# Autodesk Inventor assembly: segment2
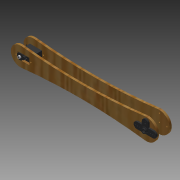
[picture p0: Inventor's stored thumbnail of the model, 180x180]
Saved by Autodesk Inventor 2013 (Build 170138000, 138)
## iProperties
Created: 2014-10-09
Part Number: segment2
Document SubType Name: Assembly
Designer: Masta
Author: Masta
## Documents named in this file (4)
- D:\DrOctopus\3D model\segment2.iam
- D:\DrOctopus\3D model\servo arm BMS-630MG tripple.ipt
- D:\DrOctopus\3D model\segment2a.ipt
- D:\DrOctopus\3D model\serwo 2.8kg DS939HV.ipt
## Components (4 placed, 3 different names)
1. servo arm BMS-630MG tripple:1 — Insert:1, Insert:2
2. segment2a:1 — Insert:1, Insert:2, Insert:3, Insert:4, Insert:5, Tangent:1
3. serwo 2.8kg DS939HV:1 — Insert:3, Insert:4
4. segment2a:2 — Insert:5, Tangent:1
## Relationships (6: Insert 5, Tangent 1)
- Insert:1: servo arm BMS-630MG tripple:1 ↔ segment2a:1
- Insert:2: servo arm BMS-630MG tripple:1 ↔ segment2a:1
- Insert:3 (2 mm): segment2a:1 ↔ serwo 2.8kg DS939HV:1
- Insert:4 (2 mm): segment2a:1 ↔ serwo 2.8kg DS939HV:1
- Insert:5 (20 mm): segment2a:1 ↔ segment2a:2
- Tangent:1: segment2a:1 ↔ segment2a:2
